# Autodesk Inventor assembly: ASY МОО 001 отстойник осветлитель
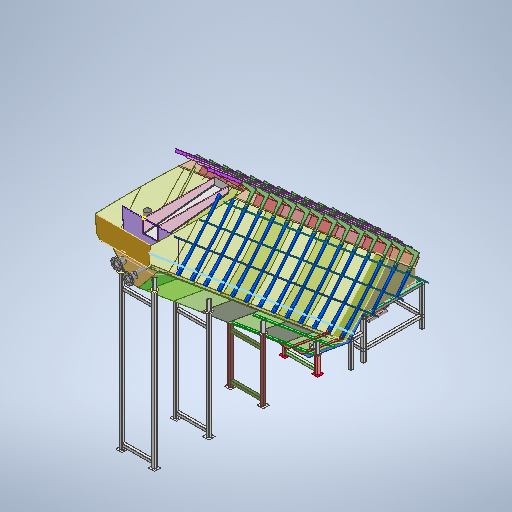
[picture p0: Inventor's stored thumbnail of the model, 512x512]
Saved by Autodesk Inventor 2025 (Build 290162010, 162A)
## iProperties
Created: 2024-04-28
Part Number: ASY МОО 001 отстойник осветлитель
Document SubType Name: Weldment
Designer: admin
Weld Material: Welded Aluminum-6061
Mass: 1.58517e+06 g
Surface Area: 1.48953e+06 cm^2
Volume: 226523 cm^3
Density: 6.99781 g/cm^3
Author: admin
## Documents named in this file (68)
- C:\Users\pokla\Documents\Inventor\Отстойник осветлитель\Manturovo_Se-clar-Gleb\ASY МОО 001 отстойник осветлитель.iam
- C:\Users\pokla\Documents\Inventor\Отстойник осветлитель\Manturovo_Se-clar-Gleb\Пример емкости.ipt
- C:\Users\pokla\Documents\Inventor\Отстойник осветлитель\Manturovo_Se-clar-Gleb\MSC 041 sheet belly main.ipt
- C:\Users\pokla\Documents\Inventor\Отстойник осветлитель\Manturovo_Se-clar-Gleb\MSC 052 rib board.ipt
- C:\Users\pokla\Documents\Inventor\Отстойник осветлитель\Manturovo_Se-clar-Gleb\Рама основания\ASY MSC 090 base frame.iam
- C:\Users\pokla\Documents\Inventor\Отстойник осветлитель\Manturovo_Se-clar-Gleb\ASY MSC 080 roсket.iam
- C:\Users\pokla\Documents\Inventor\Отстойник осветлитель\Manturovo_Se-clar-Gleb\ASY MSC 010 cone.iam
- C:\Users\pokla\Documents\Inventor\Отстойник осветлитель\Manturovo_Se-clar-Gleb\ракета\МОО 064 ракета труба.ipt
- C:\Users\pokla\Documents\Inventor\Отстойник осветлитель\Manturovo_Se-clar-Gleb\MSC 000 DIM settler-clarifier.ipt
- C:\Users\pokla\Documents\Inventor\Отстойник осветлитель\Manturovo_Se-clar-Gleb\MSC 031 sheet lowerback.ipt
- C:\Users\pokla\Documents\Inventor\Отстойник осветлитель\Manturovo_Se-clar-Gleb\MSC 024 sheet board main.ipt
- C:\Users\pokla\Documents\Inventor\Отстойник осветлитель\Manturovo_Se-clar-Gleb\MSC 021 sheet left board hip.ipt
- C:\Users\pokla\Documents\Inventor\Отстойник осветлитель\Manturovo_Se-clar-Gleb\MSC 022 sheet right board hip.ipt
- C:\Users\pokla\Documents\Inventor\Отстойник осветлитель\Manturovo_Se-clar-Gleb\MSC 042 sheet belly-neck.ipt
- C:\Users\pokla\Documents\Inventor\Отстойник осветлитель\Manturovo_Se-clar-Gleb\MSC 023 sheet board.ipt
- C:\Users\pokla\Documents\Inventor\Отстойник осветлитель\Manturovo_Se-clar-Gleb\конус\MSC 071 ridge 1.ipt
- C:\Users\pokla\Documents\Inventor\Отстойник осветлитель\Manturovo_Se-clar-Gleb\конус\MSC 073 ridge 3.ipt
- C:\Users\pokla\Documents\Inventor\Отстойник осветлитель\Manturovo_Se-clar-Gleb\конус\MSC 074 face 1.ipt
- C:\Users\pokla\Documents\Inventor\Отстойник осветлитель\Manturovo_Se-clar-Gleb\Content Center Files\en-US\ISO 5251 B 3D\ISO 5251 Bends 3D without straight ends(90 deg) DN150 11 11.ipt
- C:\Users\pokla\Documents\Inventor\Отстойник осветлитель\Manturovo_Se-clar-Gleb\Content Center Files\en-US\DIN EN 1092-1 01 - PN 25\DIN EN 1092-1 Plate Flange for Welding Type 01 - PN 25 150 x 168.3.ipt
- C:\Users\pokla\Documents\Inventor\Отстойник осветлитель\Manturovo_Se-clar-Gleb\МОО 061 труба верх 1.ipt
- C:\Users\pokla\Documents\Inventor\Отстойник осветлитель\Manturovo_Se-clar-Gleb\МОО 062 труба верх 2.ipt
- C:\Users\pokla\Documents\Inventor\Отстойник осветлитель\Manturovo_Se-clar-Gleb\МОО 063 труба верх 3.ipt
- C:\Users\pokla\Documents\Inventor\Отстойник осветлитель\Manturovo_Se-clar-Gleb\MSC 063 stringer board #.ipt
- C:\Users\pokla\Documents\Inventor\Отстойник осветлитель\Manturovo_Se-clar-Gleb\MSC 064 stringer board ##.ipt
- C:\Users\pokla\Documents\Inventor\Отстойник осветлитель\Manturovo_Se-clar-Gleb\MSC 065 stringer board ###.ipt
- C:\Users\pokla\Documents\Inventor\Отстойник осветлитель\Manturovo_Se-clar-Gleb\MSC 066 stringer board ####.ipt
- C:\Users\pokla\Documents\Inventor\Отстойник осветлитель\Manturovo_Se-clar-Gleb\MSC 067 stringer board belly.ipt
- C:\Users\pokla\Documents\Inventor\Отстойник осветлитель\Manturovo_Se-clar-Gleb\MSC 053 rib belly.ipt
- C:\Users\pokla\Documents\Inventor\Отстойник осветлитель\Manturovo_Se-clar-Gleb\Part1.ipt
- C:\Users\pokla\Documents\Inventor\Отстойник осветлитель\Manturovo_Se-clar-Gleb\стапель\ASY стапель.iam
- C:\Users\pokla\Documents\Inventor\Отстойник осветлитель\Manturovo_Se-clar-Gleb\MSC 0101 sheet gills.ipt
- C:\Users\pokla\Documents\Inventor\Отстойник осветлитель\Manturovo_Se-clar-Gleb\MSC 026 sheet board withers 2.ipt
- C:\Users\pokla\Documents\Inventor\Отстойник осветлитель\Manturovo_Se-clar-Gleb\MSC 028 sheet board face 2.ipt
- C:\Users\pokla\Documents\Inventor\Отстойник осветлитель\Manturovo_Se-clar-Gleb\MSC 068 stringer lowerback.ipt
- C:\Users\pokla\Documents\Inventor\Отстойник осветлитель\Manturovo_Se-clar-Gleb\конус\MSC 072 ridge 2.ipt
- C:\Users\pokla\Documents\Inventor\Отстойник осветлитель\Manturovo_Se-clar-Gleb\MSC 075 face 2.ipt
- C:\Users\pokla\Documents\Inventor\Отстойник осветлитель\Manturovo_Se-clar-Gleb\MSC 076 face 3.ipt
- C:\Users\pokla\Documents\Inventor\Отстойник осветлитель\Manturovo_Se-clar-Gleb\MSC 077 face 4.ipt
- C:\Users\pokla\Documents\Inventor\Отстойник осветлитель\Manturovo_Se-clar-Gleb\MSC 055 rib hip 2.ipt
- C:\Users\pokla\Documents\Inventor\Отстойник осветлитель\Manturovo_Se-clar-Gleb\MSC 110 revision hatch 1.ipt
- C:\Users\pokla\Documents\Inventor\Отстойник осветлитель\Manturovo_Se-clar-Gleb\MSC 054 rib hip 1.ipt
- C:\Users\pokla\Documents\Inventor\Отстойник осветлитель\Manturovo_Se-clar-Gleb\MSC 035 ring.ipt
- C:\Users\pokla\Documents\Inventor\Отстойник осветлитель\Manturovo_Se-clar-Gleb\MSC 074 ridge 4.ipt
- C:\Users\pokla\Documents\Inventor\Отстойник осветлитель\Manturovo_Se-clar-Gleb\MSC 075 ridge 5.ipt
- C:\Users\pokla\Documents\Inventor\Отстойник осветлитель\Manturovo_Se-clar-Gleb\MSC 081 pillar 1.ipt
- C:\Users\pokla\Documents\Inventor\Отстойник осветлитель\Manturovo_Se-clar-Gleb\MSC 036 flange 500.ipt
- C:\Users\pokla\Documents\Inventor\Отстойник осветлитель\Manturovo_Se-clar-Gleb\MSC 037 flange cover 500.ipt
- C:\Users\pokla\Documents\Inventor\Отстойник осветлитель\Manturovo_Se-clar-Gleb\MSC 038 flange cover ring 500.ipt
- C:\Users\pokla\Documents\Inventor\Отстойник осветлитель\Manturovo_Se-clar-Gleb\MSC 039 flange cover plate 500.ipt
- C:\Users\pokla\Documents\Inventor\Отстойник осветлитель\Manturovo_Se-clar-Gleb\Content Center Files\en-US\DIN EN ISO 8676\DIN EN ISO 8676 - M12 x 1,5 x 30.ipt
- C:\Users\pokla\Documents\Inventor\Отстойник осветлитель\Manturovo_Se-clar-Gleb\Content Center Files\en-US\ISO 4032(2)\ISO 4032 - M12 - ISO.ipt
- C:\Users\pokla\Documents\Inventor\Отстойник осветлитель\Manturovo_Se-clar-Gleb\Рама основания\ASY MSC 120  base frame.iam
- C:\Users\pokla\Documents\Inventor\Отстойник осветлитель\Manturovo_Se-clar-Gleb\Рама основания\ASY MSC 121  base frame.iam
- C:\Users\pokla\Documents\Inventor\Отстойник осветлитель\Manturovo_Se-clar-Gleb\Чертеж для парам. рамы.ipt
- C:\Users\pokla\Documents\Inventor\Отстойник осветлитель\Manturovo_Se-clar-Gleb\ASY MSC 120.1  base frame.iam
- C:\Users\pokla\Documents\Inventor\Отстойник осветлитель\Manturovo_Se-clar-Gleb\ASY MSC 122  base frame.iam
- C:\Users\pokla\Documents\Inventor\Отстойник осветлитель\Manturovo_Se-clar-Gleb\ASY MSC 123  base frame.iam
- C:\Users\pokla\Documents\Inventor\Отстойник осветлитель\Manturovo_Se-clar-Gleb\ASY MSC 124  base frame.iam
- C:\Users\pokla\Documents\Inventor\Отстойник осветлитель\Manturovo_Se-clar-Gleb\MSC 125 base tube.ipt
- C:\Users\pokla\Documents\Inventor\Отстойник осветлитель\Manturovo_Se-clar-Gleb\MSC 126 flange base tube.ipt
- C:\Users\pokla\Documents\Inventor\Отстойник осветлитель\Manturovo_Se-clar-Gleb\MSC 128 flange base tube support.ipt
- C:\Users\pokla\Documents\Inventor\Отстойник осветлитель\Manturovo_Se-clar-Gleb\MSC 125 base tube_MIR2.ipt
- C:\Users\pokla\Documents\Inventor\Отстойник осветлитель\Manturovo_Se-clar-Gleb\DXF файлы\MSC 126 flange base tube_MIR2.ipt
- C:\Users\pokla\Documents\Inventor\Отстойник осветлитель\Manturovo_Se-clar-Gleb\DXF файлы\MSC 128 flange base tube support_MIR1.ipt
- C:\Users\pokla\Documents\Inventor\Отстойник осветлитель\Manturovo_Se-clar-Gleb\MSC 0512 rib back mould .ipt
- C:\Users\pokla\Documents\Inventor\Отстойник осветлитель\Manturovo_Se-clar-Gleb\ASY MSC 201 BACK.iam
- C:\Users\pokla\Documents\Inventor\Отстойник осветлитель\Manturovo_Se-clar-Gleb\ASY MSC 202 LEFT BOARD.iam
## Components (129 placed, 68 different names)
1. Пример емкости.ipt:1 — Mate:1, Mate:2, Flush:2
2. MSC 000 DIM settler-clarifier.ipt:1
3. ASY MSC 090 base frame.iam:1 [sub-assembly] — Flush:19, Flush:21, Flush:82, Mate:82
4. ASY MSC 010 cone.iam:1 [sub-assembly] — Flush:22, Mate:16, Flush:28, Mate:54, Mate:57, Mate:65, Mate:78, Tangent:11, Flush:79, Mate:82, Mate:83
5. MSC 041 sheet belly main.ipt:1 — Mate:9, Rigid:18, Rigid:40
6. ASY MSC 080 roсket.iam:1 [sub-assembly] — Flush:23
7. МОО 064 ракета труба.ipt:1
8. MSC 031 sheet lowerback.ipt:1 — Mate:15, Mate:16, Tangent:10, Tangent:11, Tangent:12, Cylindrical:2, Rigid:185
9. MSC 041 sheet belly main.ipt:2 — Rigid:18, Rigid:53
10. MSC 021 sheet left board hip.ipt:1 — Flush:41, Mate:78
11. MSC 022 sheet right board hip.ipt:1 — Mate:30
12. MSC 041 sheet belly main.ipt:3 — Rigid:40, Rigid:47
13. MSC 042 sheet belly-neck.ipt:1 — Rigid:48, Mate:70, Mate:71
14. MSC 041 sheet belly main.ipt:4 — Rigid:45, Rigid:47
15. MSC 041 sheet belly main.ipt:5 — Rigid:45, Rigid:48
16. MSC 071 ridge 1.ipt:1 — Mate:50, Flush:57, Mate:68, Flush:81, Flush:83, Mate:85
17. MSC 074 face 1.ipt:1 — Rigid:156, Rigid:157, Mate:70, Flush:62, Mate:71, Rigid:159, Mate:80
18. MSC 041 sheet belly main.ipt:6 — Mate:54, Rigid:53, Mate:93, Mate:96
19. MSC 073 ridge 3.ipt:1 — Flush:57, Mate:68, Mate:77, Flush:78, Mate:81, Flush:80
20. DIN EN 1092-1 Plate Flange for Welding Type 01 - PN 25 150 x 168.3.ipt:1 — Rigid:158
21. МОО 061 труба верх 1.ipt:1 — Rigid:158, Rigid:59, Rigid:159
22. ISO 5251 Bends 3D without straight ends(90 deg) DN150 11 11.ipt:1 — Rigid:59, Rotational:2
23. МОО 062 труба верх 2.ipt:1 — Rigid:132, Rigid:156
24. DIN EN 1092-1 Plate Flange for Welding Type 01 - PN 25 150 x 168.3.ipt:2 — Rigid:132
25. МОО 063 труба верх 3.ipt:1 — Rigid:157
26. MSC 024 sheet board main.ipt:6 — Rigid:134
27. MSC 024 sheet board main.ipt:7
28. MSC 024 sheet board main.ipt:8
29. MSC 024 sheet board main.ipt:9
30. MSC 024 sheet board main.ipt:10 — Rigid:67
31. MSC 023 sheet board.ipt:2 — Rigid:67, Mate:57, Mate:58
32. MSC 052 rib board.ipt:1 — Rigid:161, Rigid:162, Rigid:163, Rigid:164
33. MSC 066 stringer board ####.ipt:1 — Rigid:143, Rigid:162
34. MSC 065 stringer board ###.ipt:1 — Rigid:142, Rigid:163
35. MSC 064 stringer board ##.ipt:1 — Rigid:141, Rigid:164
36. MSC 063 stringer board #.ipt:1 — Rigid:140
37. Part1.ipt:1
38. ASY стапель.iam:1 [sub-assembly] — Mate:63
39. MSC 053 rib belly.ipt:2 — Rigid:110, Rigid:126, Rigid:127
40. MSC 053 rib belly.ipt:1 — Rigid:111, Rigid:112, Rigid:127
41. MSC 067 stringer board belly.ipt:4 — Rigid:126, Rigid:147
42. MSC 067 stringer board belly.ipt:3 — Rigid:110, Rigid:146
43. MSC 067 stringer board belly.ipt:2 — Rigid:112, Rigid:144
44. MSC 067 stringer board belly.ipt:1 — Rigid:111, Rigid:145
45. MSC 0101 sheet gills.ipt:1 — Mate:64
46. MSC 026 sheet board withers 2.ipt:1 — Rigid:133, Rigid:134
47. MSC 028 sheet board face 2.ipt:1 — Rigid:133
48. MSC 068 stringer lowerback.ipt:1 — Mate:65, Tangent:10
49. MSC 053 rib belly.ipt:4
50. MSC 052 rib board.ipt:4
51. MSC 053 rib belly.ipt:3
52. MSC 067 stringer board belly.ipt:8 — Rigid:144
53. MSC 067 stringer board belly.ipt:7 — Rigid:145
54. MSC 066 stringer board ####.ipt:4 — Rigid:143
55. MSC 065 stringer board ###.ipt:4 — Rigid:142
56. MSC 064 stringer board ##.ipt:4 — Rigid:141
57. MSC 063 stringer board #.ipt:4 — Rigid:140, Rigid:161
58. MSC 067 stringer board belly.ipt:6 — Rigid:146
59. MSC 067 stringer board belly.ipt:5 — Rigid:147
60. MSC 072 ridge 2.ipt:1 — Flush:58, Mate:81, Flush:80, Flush:81, Flush:84
61. МОО 061 труба верх 1.ipt:2 — Rotational:2
62. MSC 075 face 2.ipt:1 — Flush:61, Mate:76
63. MSC 076 face 3.ipt:1 — Flush:76, Mate:76
64. MSC 077 face 4.ipt:1 — Mate:77, Flush:77, Flush:78, Mate:80
65. MSC 110 revision hatch 1:1 — Flush:82
66. MSC 055 rib hip 2:2
67. MSC 054 rib board hip 1:2
68. MSC 068 stringer lowerback:2 — Mate:83, Tangent:12
69. MSC 035 ring:1 — Cylindrical:2, Rigid:185, Rigid:186
70. MSC 074 ridge 4:1 — Flush:83, Mate:85, Flush:84, Rigid:173
71. MSC 075 ridge 5:1 — Rigid:173
72. MSC 081 pillar 1:1 — Insert:1, Insert:2, Insert:3, Insert:4, Rigid:179, Mate:93
73. MSC 036 flange 500:1 — Rigid:175
74. MSC 036 flange 500:2 — Rigid:175, Rigid:176, Rigid:186
75. MSC 036 flange 500:3 — Rigid:176, Rigid:177, Mate:87
76. MSC 036 flange 500:4 — Rigid:177, Rotational:4
77. MSC 037 flange cover 500:1 — Rotational:4, Mate:87, Rigid:178, Mate:108
78. MSC 038 flange cover ring 500:1 — Rigid:178, Mate:109, Tangent:15
79. DIN EN ISO 8676 M12 x 1,5 x 30:1 — Rigid:179
80. ISO 4032 M12:1 — Insert:2
81. ISO 4032 M12:2 — Insert:1
82. ISO 4032 M12:3 — Insert:3
83. ISO 4032 M12:4 — Insert:4
84. ASY MSC 120  base frame:1 [sub-assembly] — Flush:93, Mate:97, Rotational:5
85. ASY MSC 121  base frame:1 [sub-assembly] — Mate:98, Flush:95, Mate:99
86. Чертеж для парам. рамы:1 — Flush:94, Mate:95, Mate:96, Mate:97, Mate:99, Mate:100, Mate:103, Mate:105, Mate:107
87. ASY MSC 120.1  base frame:2 [sub-assembly] — Flush:96, Mate:100, Mate:101
88. ASY MSC 122  base frame:2 [sub-assembly] — Flush:97, Mate:102, Mate:103
89. ASY MSC 123  base frame:2 [sub-assembly] — Flush:98, Mate:104, Mate:105
90. ASY MSC 124  base frame:2 [sub-assembly] — Flush:99, Mate:106, Mate:107
91. MSC 0512 rib back mould :1
92. ASY MSC 201 BACK:1 [sub-assembly] — Mate:110
93. ASY MSC 202 LEFT BOARD:1 [sub-assembly]
94. MSC 126 flange base tube_MIR2:1 — Rigid:183
95. MSC 125 base tube_MIR2:1 — Rigid:183, Rigid:184
96. MSC 128 flange base tube support_MIR1:1 — Rigid:184
97. MSC 125 base tube:1 — Rigid:180, Rigid:182
98. MSC 128 flange base tube support:1 — Rigid:182
99. MSC 126 flange base tube:1 — Rigid:180, Rotational:5
100. MSC 126 flange base tube_MIR2:2
101. MSC 125 base tube_MIR2:2
102. MSC 128 flange base tube support_MIR1:2
103. MSC 125 base tube:2
104. MSC 128 flange base tube support:2
105. MSC 126 flange base tube:2
106. MSC 126 flange base tube_MIR2:3
107. MSC 125 base tube_MIR2:3
108. MSC 128 flange base tube support_MIR1:3
109. MSC 125 base tube:3
110. MSC 128 flange base tube support:3
111. MSC 126 flange base tube:3
112. MSC 126 flange base tube_MIR2:4
113. MSC 125 base tube_MIR2:4
114. MSC 128 flange base tube support_MIR1:4
115. MSC 125 base tube:4
116. MSC 128 flange base tube support:4
117. MSC 126 flange base tube:4
118. MSC 039 flange cover plate 500:1 — Mate:108, Mate:109, Tangent:15
119. MSC 039 flange cover plate 500:2
120. MSC 039 flange cover plate 500:3
121. MSC 039 flange cover plate 500:4
122. MSC 039 flange cover plate 500:5
123. MSC 039 flange cover plate 500:6
124. MSC 039 flange cover plate 500:7
125. MSC 039 flange cover plate 500:8
126. MSC 039 flange cover plate 500:9
127. MSC 039 flange cover plate 500:10
128. MSC 039 flange cover plate 500:11
129. MSC 039 flange cover plate 500:12
## Component patterns: (4 elements, first: MSC 126 flange base tube_MIR2:1 + MSC 125 base tube_MIR2:1 + MSC 128 flange base tube support_MIR1:1 + MSC 125 base tube:1 + MSC 128 flange base tube support:1 + MSC 126 flange base tube:1), (12 elements, first: MSC 039 flange cover plate 500:1)
## Relationships (169: WeldJoint 57, Mate 54, Flush 41, Tangent 9, Insert 4, RevoluteJoint 3, CylindricalJoint 1)
- Mate:1: Пример емкости.ipt:1
- Mate:2: Пример емкости.ipt:1
- Flush:2: Пример емкости.ipt:1
- [Flush]: ASY MSC 201 BACK:1
- Mate:9: MSC 041 sheet belly main.ipt:1
- [Flush]: ASY MSC 201 BACK:1
- Flush:19: ASY MSC 090 base frame.iam:1
- Flush:21: ASY MSC 090 base frame.iam:1
- Flush:22: ASY MSC 010 cone.iam:1
- Flush:23: ASY MSC 080 roсket.iam:1
- Mate:15: MSC 031 sheet lowerback.ipt:1
- [Flush]: ASY MSC 201 BACK:1
- Mate:16: ASY MSC 010 cone.iam:1 ↔ MSC 031 sheet lowerback.ipt:1
- Flush:28: ASY MSC 010 cone.iam:1
- [Flush]: ASY MSC 202 LEFT BOARD:1
- [Tangent]: ASY MSC 201 BACK:1 ↔ ASY MSC 202 LEFT BOARD:1
- Rigid:18 [WeldJoint]: MSC 041 sheet belly main.ipt:1 ↔ MSC 041 sheet belly main.ipt:2
- [Mate]: ASY MSC 201 BACK:1
- Flush:41: MSC 021 sheet left board hip.ipt:1
- [Flush]: MSC 021 sheet left board hip.ipt:1 ↔ ASY MSC 201 BACK:1
- [Tangent]: MSC 021 sheet left board hip.ipt:1 ↔ ASY MSC 201 BACK:1
- Mate:30: MSC 022 sheet right board hip.ipt:1
- [Flush]: MSC 022 sheet right board hip.ipt:1 ↔ ASY MSC 201 BACK:1
- [Tangent]: MSC 022 sheet right board hip.ipt:1 ↔ ASY MSC 201 BACK:1
- [Mate]: ASY MSC 010 cone.iam:1 ↔ ASY MSC 201 BACK:1
- Rigid:40 [WeldJoint]: MSC 041 sheet belly main.ipt:1 ↔ MSC 041 sheet belly main.ipt:3
- Rigid:45 [WeldJoint]: MSC 041 sheet belly main.ipt:4 ↔ MSC 041 sheet belly main.ipt:5
- Rigid:47 [WeldJoint]: MSC 041 sheet belly main.ipt:3 ↔ MSC 041 sheet belly main.ipt:4
- Rigid:48 [WeldJoint]: MSC 042 sheet belly-neck.ipt:1 ↔ MSC 041 sheet belly main.ipt:5
- [Mate]: ASY MSC 010 cone.iam:1 ↔ ASY MSC 202 LEFT BOARD:1
- [Flush]: ASY MSC 202 LEFT BOARD:1
- [Tangent]: ASY MSC 201 BACK:1 ↔ ASY MSC 202 LEFT BOARD:1
- Mate:50 (200 mm): MSC 071 ridge 1.ipt:1
- Mate:54: ASY MSC 010 cone.iam:1 ↔ MSC 041 sheet belly main.ipt:6
- [Mate]: MSC 041 sheet belly main.ipt:6 ↔ ASY MSC 202 LEFT BOARD:1
- Rigid:53 [WeldJoint]: MSC 041 sheet belly main.ipt:2 ↔ MSC 041 sheet belly main.ipt:6
- Rigid:158 [WeldJoint]: DIN EN 1092-1 Plate Flange for Welding Type 01 - PN 25 150 x 168.3.ipt:1 ↔ МОО 061 труба верх 1.ipt:1
- Rigid:59 [WeldJoint]: МОО 061 труба верх 1.ipt:1 ↔ ISO 5251 Bends 3D without straight ends(90 deg) DN150 11 11.ipt:1
- [WeldJoint]: MSC 024 sheet board main.ipt:6 ↔ MSC 024 sheet board main.ipt:7
- [WeldJoint]: MSC 024 sheet board main.ipt:7 ↔ MSC 024 sheet board main.ipt:8
- [WeldJoint]: MSC 024 sheet board main.ipt:8 ↔ MSC 024 sheet board main.ipt:9
- [WeldJoint]: MSC 024 sheet board main.ipt:9 ↔ MSC 024 sheet board main.ipt:10
- Rigid:67 [WeldJoint]: MSC 024 sheet board main.ipt:10 ↔ MSC 023 sheet board.ipt:2
- Mate:57: ASY MSC 010 cone.iam:1 ↔ MSC 023 sheet board.ipt:2
- Mate:58: MSC 023 sheet board.ipt:2
- [Tangent]: MSC 023 sheet board.ipt:2 ↔ ASY MSC 201 BACK:1
- [WeldJoint] (-50 mm): ASY MSC 201 BACK:1 ↔ ASY MSC 202 LEFT BOARD:1
- [WeldJoint] (-50 mm): MSC 052 rib board.ipt:1 ↔ ASY MSC 201 BACK:1
- Rigid:110 [WeldJoint] (2 mm): MSC 053 rib belly.ipt:2 ↔ MSC 067 stringer board belly.ipt:3
- Rigid:111 [WeldJoint] (2 mm): MSC 053 rib belly.ipt:1 ↔ MSC 067 stringer board belly.ipt:1
- Rigid:112 [WeldJoint] (2 mm): MSC 053 rib belly.ipt:1 ↔ MSC 067 stringer board belly.ipt:2
- [Flush]: MSC 053 rib belly.ipt:2 ↔ ASY MSC 202 LEFT BOARD:1
- [Flush]: MSC 053 rib belly.ipt:2 ↔ ASY MSC 202 LEFT BOARD:1
- Rigid:126 [WeldJoint] (2 mm): MSC 053 rib belly.ipt:2 ↔ MSC 067 stringer board belly.ipt:4
- [Mate]: MSC 053 rib belly.ipt:2 ↔ ASY MSC 202 LEFT BOARD:1
- [Mate]: ASY стапель.iam:1 ↔ ASY MSC 201 BACK:1
- [Flush]: ASY стапель.iam:1 ↔ ASY MSC 201 BACK:1
- Mate:63: ASY стапель.iam:1
- Rigid:127 [WeldJoint] (-50 mm): MSC 053 rib belly.ipt:2 ↔ MSC 053 rib belly.ipt:1
- Rigid:132 [WeldJoint]: МОО 062 труба верх 2.ipt:1 ↔ DIN EN 1092-1 Plate Flange for Welding Type 01 - PN 25 150 x 168.3.ipt:2
- Mate:64: MSC 0101 sheet gills.ipt:1
- Rigid:133 [WeldJoint]: MSC 026 sheet board withers 2.ipt:1 ↔ MSC 028 sheet board face 2.ipt:1
- Rigid:134 [WeldJoint]: MSC 024 sheet board main.ipt:6 ↔ MSC 026 sheet board withers 2.ipt:1
- Mate:65: ASY MSC 010 cone.iam:1 ↔ MSC 068 stringer lowerback.ipt:1
- [Mate]: MSC 068 stringer lowerback.ipt:1 ↔ ASY MSC 201 BACK:1
- Tangent:10: MSC 031 sheet lowerback.ipt:1 ↔ MSC 068 stringer lowerback.ipt:1
- [WeldJoint] (-50 mm): ASY MSC 201 BACK:1 ↔ ASY MSC 202 LEFT BOARD:1
- [WeldJoint] (-50 mm): MSC 052 rib board.ipt:4 ↔ ASY MSC 201 BACK:1
- [Flush]: MSC 053 rib belly.ipt:4 ↔ ASY MSC 202 LEFT BOARD:1
- [Flush]: MSC 053 rib belly.ipt:4 ↔ ASY MSC 202 LEFT BOARD:1
- [Mate]: MSC 053 rib belly.ipt:4 ↔ ASY MSC 202 LEFT BOARD:1
- [WeldJoint] (-50 mm): MSC 053 rib belly.ipt:4 ↔ MSC 053 rib belly.ipt:3
- Rigid:140 [WeldJoint] (2 mm): MSC 063 stringer board #.ipt:1 ↔ MSC 063 stringer board #.ipt:4
- Rigid:141 [WeldJoint]: MSC 064 stringer board ##.ipt:1 ↔ MSC 064 stringer board ##.ipt:4
- Rigid:142 [WeldJoint]: MSC 065 stringer board ###.ipt:1 ↔ MSC 065 stringer board ###.ipt:4
- Rigid:143 [WeldJoint]: MSC 066 stringer board ####.ipt:1 ↔ MSC 066 stringer board ####.ipt:4
- Rigid:144 [WeldJoint]: MSC 067 stringer board belly.ipt:2 ↔ MSC 067 stringer board belly.ipt:8
- Rigid:145 [WeldJoint]: MSC 067 stringer board belly.ipt:1 ↔ MSC 067 stringer board belly.ipt:7
- Rigid:146 [WeldJoint]: MSC 067 stringer board belly.ipt:3 ↔ MSC 067 stringer board belly.ipt:6
- Rigid:147 [WeldJoint]: MSC 067 stringer board belly.ipt:4 ↔ MSC 067 stringer board belly.ipt:5
- [Flush] (200 mm): MSC 073 ridge 3.ipt:1 ↔ ASY MSC 202 LEFT BOARD:1
- Flush:57: MSC 071 ridge 1.ipt:1 ↔ MSC 073 ridge 3.ipt:1
- Mate:68: MSC 071 ridge 1.ipt:1 ↔ MSC 073 ridge 3.ipt:1
- Flush:58 (200 mm): MSC 072 ridge 2.ipt:1
- Rotational:2 [RevoluteJoint]: ISO 5251 Bends 3D without straight ends(90 deg) DN150 11 11.ipt:1 ↔ МОО 061 труба верх 1.ipt:2
- [Mate]: MSC 075 face 2.ipt:1 ↔ ASY MSC 202 LEFT BOARD:1
- [Flush]: MSC 075 face 2.ipt:1 ↔ ASY MSC 202 LEFT BOARD:1
- Flush:61: MSC 075 face 2.ipt:1
- Rigid:156 [WeldJoint]: MSC 074 face 1.ipt:1 ↔ МОО 062 труба верх 2.ipt:1
- Rigid:157 [WeldJoint]: MSC 074 face 1.ipt:1 ↔ МОО 063 труба верх 3.ipt:1
- Mate:70: MSC 042 sheet belly-neck.ipt:1 ↔ MSC 074 face 1.ipt:1
- Flush:62: MSC 074 face 1.ipt:1
- Mate:71: MSC 042 sheet belly-neck.ipt:1 ↔ MSC 074 face 1.ipt:1
- Rigid:159 [WeldJoint] (-200 mm): MSC 074 face 1.ipt:1 ↔ МОО 061 труба верх 1.ipt:1
- Flush:76: MSC 076 face 3.ipt:1
- [Mate]: MSC 076 face 3.ipt:1 ↔ ASY MSC 202 LEFT BOARD:1
- Mate:76: MSC 075 face 2.ipt:1 ↔ MSC 076 face 3.ipt:1
- Mate:77: MSC 073 ridge 3.ipt:1 ↔ MSC 077 face 4.ipt:1
- Flush:77: MSC 077 face 4.ipt:1
- Flush:78: MSC 073 ridge 3.ipt:1 ↔ MSC 077 face 4.ipt:1
- Mate:78: ASY MSC 010 cone.iam:1 ↔ MSC 021 sheet left board hip.ipt:1
- Tangent:11 (22 mm): ASY MSC 010 cone.iam:1 ↔ MSC 031 sheet lowerback.ipt:1
- Flush:79: ASY MSC 010 cone.iam:1
- Rigid:161 [WeldJoint] (2 mm): MSC 052 rib board.ipt:1 ↔ MSC 063 stringer board #.ipt:4
- Rigid:162 [WeldJoint] (2 mm): MSC 052 rib board.ipt:1 ↔ MSC 066 stringer board ####.ipt:1
- Rigid:163 [WeldJoint] (2 mm): MSC 052 rib board.ipt:1 ↔ MSC 065 stringer board ###.ipt:1
- Rigid:164 [WeldJoint] (2 mm): MSC 052 rib board.ipt:1 ↔ MSC 064 stringer board ##.ipt:1
- Mate:80: MSC 074 face 1.ipt:1 ↔ MSC 077 face 4.ipt:1
- Mate:81: MSC 073 ridge 3.ipt:1 ↔ MSC 072 ridge 2.ipt:1
- Flush:80: MSC 073 ridge 3.ipt:1 ↔ MSC 072 ridge 2.ipt:1
- Flush:81: MSC 071 ridge 1.ipt:1 ↔ MSC 072 ridge 2.ipt:1
- [WeldJoint] (-50 mm): ASY MSC 201 BACK:1 ↔ ASY MSC 202 LEFT BOARD:1
- Flush:82: ASY MSC 090 base frame.iam:1 ↔ MSC 110 revision hatch 1:1
- Mate:82: ASY MSC 090 base frame.iam:1 ↔ ASY MSC 010 cone.iam:1
- [WeldJoint] (-50 mm): ASY MSC 201 BACK:1 ↔ ASY MSC 202 LEFT BOARD:1
- [WeldJoint] (-50 mm): MSC 055 rib hip 2:2 ↔ ASY MSC 201 BACK:1
- [WeldJoint] (-50 mm): MSC 054 rib board hip 1:2 ↔ ASY MSC 201 BACK:1
- Mate:83: ASY MSC 010 cone.iam:1 ↔ MSC 068 stringer lowerback:2
- [Mate]: MSC 068 stringer lowerback:2 ↔ ASY MSC 201 BACK:1
- Tangent:12: MSC 031 sheet lowerback.ipt:1 ↔ MSC 068 stringer lowerback:2
- Flush:83: MSC 071 ridge 1.ipt:1 ↔ MSC 074 ridge 4:1
- Mate:85: MSC 071 ridge 1.ipt:1 ↔ MSC 074 ridge 4:1
- Flush:84: MSC 072 ridge 2.ipt:1 ↔ MSC 074 ridge 4:1
- Rigid:173 [WeldJoint]: MSC 074 ridge 4:1 ↔ MSC 075 ridge 5:1
- Rigid:175 [WeldJoint]: MSC 036 flange 500:1 ↔ MSC 036 flange 500:2
- Rigid:176 [WeldJoint]: MSC 036 flange 500:2 ↔ MSC 036 flange 500:3
- Rigid:177 [WeldJoint]: MSC 036 flange 500:3 ↔ MSC 036 flange 500:4
- Cylindrical:2: MSC 031 sheet lowerback.ipt:1 ↔ MSC 035 ring:1
- Rotational:4 [RevoluteJoint]: MSC 036 flange 500:4 ↔ MSC 037 flange cover 500:1
- Mate:87: MSC 036 flange 500:3 ↔ MSC 037 flange cover 500:1
- Rigid:178 [WeldJoint]: MSC 037 flange cover 500:1 ↔ MSC 038 flange cover ring 500:1
- Insert:1: MSC 081 pillar 1:1 ↔ ISO 4032 M12:2
- Insert:2: MSC 081 pillar 1:1 ↔ ISO 4032 M12:1
- Insert:3: MSC 081 pillar 1:1 ↔ ISO 4032 M12:3
- Insert:4: MSC 081 pillar 1:1 ↔ ISO 4032 M12:4
- Rigid:179 [WeldJoint] (-3 mm): MSC 081 pillar 1:1 ↔ DIN EN ISO 8676 M12 x 1,5 x 30:1
- Flush:93 (-3 mm): ASY MSC 120  base frame:1
- [Mate]: ASY MSC 120  base frame:1
- Mate:93: MSC 041 sheet belly main.ipt:6 ↔ MSC 081 pillar 1:1
- Flush:94: Чертеж для парам. рамы:1
- Mate:95: Чертеж для парам. рамы:1
- Mate:96: MSC 041 sheet belly main.ipt:6 ↔ Чертеж для парам. рамы:1
- Mate:97: ASY MSC 120  base frame:1 ↔ Чертеж для парам. рамы:1
- Mate:98: ASY MSC 121  base frame:1
- Flush:95 (-3 mm): ASY MSC 121  base frame:1
- Mate:99: ASY MSC 121  base frame:1 ↔ Чертеж для парам. рамы:1
- Flush:96 (-3 mm): ASY MSC 120.1  base frame:2
- Mate:100: Чертеж для парам. рамы:1 ↔ ASY MSC 120.1  base frame:2
- Mate:101: ASY MSC 120.1  base frame:2
- Flush:97 (-3 mm): ASY MSC 122  base frame:2
- Mate:102: ASY MSC 122  base frame:2
- Mate:103: Чертеж для парам. рамы:1 ↔ ASY MSC 122  base frame:2
- Flush:98 (-3 mm): ASY MSC 123  base frame:2
- Mate:104: ASY MSC 123  base frame:2
- Mate:105: Чертеж для парам. рамы:1 ↔ ASY MSC 123  base frame:2
- Flush:99 (-3 mm): ASY MSC 124  base frame:2
- Mate:106: ASY MSC 124  base frame:2
- Mate:107: Чертеж для парам. рамы:1 ↔ ASY MSC 124  base frame:2
- Rigid:180 [WeldJoint]: MSC 125 base tube:1 ↔ MSC 126 flange base tube:1
- Rotational:5 [RevoluteJoint]: ASY MSC 120  base frame:1 ↔ MSC 126 flange base tube:1
- Rigid:182 [WeldJoint]: MSC 125 base tube:1 ↔ MSC 128 flange base tube support:1
- Rigid:183 [WeldJoint]: MSC 126 flange base tube_MIR2:1 ↔ MSC 125 base tube_MIR2:1
- Rigid:184 [WeldJoint]: MSC 125 base tube_MIR2:1 ↔ MSC 128 flange base tube support_MIR1:1
- Mate:110: ASY MSC 201 BACK:1
- Rigid:185 [WeldJoint] (20 mm): MSC 031 sheet lowerback.ipt:1 ↔ MSC 035 ring:1
- Mate:108: MSC 037 flange cover 500:1 ↔ MSC 039 flange cover plate 500:1
- Mate:109: MSC 038 flange cover ring 500:1 ↔ MSC 039 flange cover plate 500:1
- Tangent:15: MSC 038 flange cover ring 500:1 ↔ MSC 039 flange cover plate 500:1
- Rigid:186 [WeldJoint]: MSC 035 ring:1 ↔ MSC 036 flange 500:2
## Named parameters: Бак_нахлест_фланца = 25 mm, d230_d194 = 0 mm, d231_d195 = 0 mm, d232_d160 = 0 mm, d233_d161 = 0 mm, d384_d346 = 0 mm, d385_d359 = -50 mm, d386_d341 = 0 mm, d387_d342 = 0 mm, d388_d243 = -50 mm, d389_d246 = -50 mm, Шаг_опор_по_баку = 2000 mm
